# Autodesk Inventor assembly: Slider Assembly
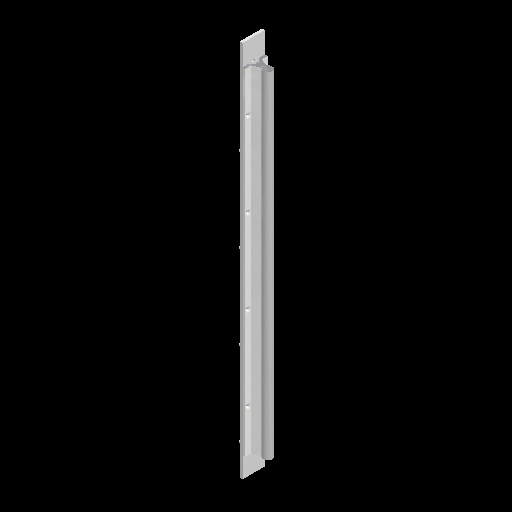
[picture p0: Inventor's stored thumbnail of the model, 512x512]
Saved by Autodesk Inventor 2026.1 (Build 301233000, 233)
## iProperties
Created: 2024-12-30
Part Number: Slider Assembly
Document SubType Name: Assembly
Designer: drago
Author: drago
## Documents named in this file (4)
- C:\Users\drago\Desktop\_QIST4500_Multidisciplinary_Team_Project\Proteox MX magnet positioner CAD\z_rail\z_rail.iam
- C:\Users\drago\Desktop\_QIST4500_Multidisciplinary_Team_Project\Proteox MX magnet positioner CAD\z_rail\item_61953_t-slot-slider-8-80x40-fa__high.ipt
- C:\Users\drago\Desktop\_QIST4500_Multidisciplinary_Team_Project\Proteox MX magnet positioner CAD\z_rail\Rail_bracket.ipt
- C:\Users\drago\Desktop\_QIST4500_Multidisciplinary_Team_Project\Proteox MX magnet positioner CAD\z_rail\SBR16_600mm.ipt
## Components (6 placed, 3 different names)
1. item_61953_t-slot-slider-8-80x40-fa__high:3 — Mate:6, Mate:8, Mate:13
2. item_61953_t-slot-slider-8-80x40-fa__high:4 — Mate:5, Mate:10, Mate:12
3. item_61953_t-slot-slider-8-80x40-fa__high:1 — Mate:1, Mate:2, Mate:11
4. Rail_bracket:1 — Mate:1, Mate:2, Mate:3, Mate:4, Mate:5, Mate:6, Mate:7, Mate:8, Mate:9, Mate:10, Mate:15, Mate:16, Mate:17
5. SBR16_600mm:1 — Mate:15, Mate:16, Mate:17
6. item_61953_t-slot-slider-8-80x40-fa__high:6 — Mate:7, Mate:9, Mate:14
## Relationships (17: Mate 17)
- Mate:1: item_61953_t-slot-slider-8-80x40-fa__high:1 ↔ Rail_bracket:1
- Mate:2: item_61953_t-slot-slider-8-80x40-fa__high:1 ↔ Rail_bracket:1
- Mate:3: Rail_bracket:1
- Mate:4: Rail_bracket:1
- Mate:5: item_61953_t-slot-slider-8-80x40-fa__high:4 ↔ Rail_bracket:1
- Mate:6: item_61953_t-slot-slider-8-80x40-fa__high:3 ↔ Rail_bracket:1
- Mate:7: Rail_bracket:1 ↔ item_61953_t-slot-slider-8-80x40-fa__high:6
- Mate:8: item_61953_t-slot-slider-8-80x40-fa__high:3 ↔ Rail_bracket:1
- Mate:9: Rail_bracket:1 ↔ item_61953_t-slot-slider-8-80x40-fa__high:6
- Mate:10: item_61953_t-slot-slider-8-80x40-fa__high:4 ↔ Rail_bracket:1
- Mate:11: item_61953_t-slot-slider-8-80x40-fa__high:1
- Mate:12: item_61953_t-slot-slider-8-80x40-fa__high:4
- Mate:13: item_61953_t-slot-slider-8-80x40-fa__high:3
- Mate:14: item_61953_t-slot-slider-8-80x40-fa__high:6
- Mate:15: Rail_bracket:1 ↔ SBR16_600mm:1
- Mate:16: Rail_bracket:1 ↔ SBR16_600mm:1
- Mate:17: Rail_bracket:1 ↔ SBR16_600mm:1
